# Autodesk Inventor assembly: field_both_side
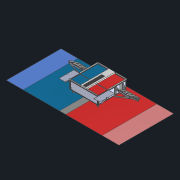
[picture p0: Inventor's stored thumbnail of the model, 180x180]
Saved by Autodesk Inventor 2022 (Build 260153000, 153)
## iProperties
Created: 2021-11-03
Part Number: field_both_side
Document SubType Name: Assembly
Designer: Yuta Kage
Author: Yuta Kage
## Documents named in this file (2)
- C:\Users\yuta0\Documents\GitHub\catchrobo_hardware\mesh\base\field_both_side.iam
- C:\Users\yuta0\Documents\GitHub\catchrobo_hardware\mesh\base\full_origin.ipt
## Components (1 placed, 1 different names)
1. full_origin:1 — フラッシュ:1, フラッシュ:2, フラッシュ:3
## Relationships (3: Flush 3)
- フラッシュ:1 [Flush]: full_origin:1
- フラッシュ:2 [Flush]: full_origin:1
- フラッシュ:3 [Flush]: full_origin:1
